# Autodesk Inventor assembly: Łapa
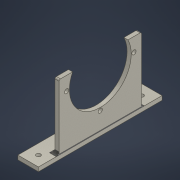
[picture p0: Inventor's stored thumbnail of the model, 180x180]
Saved by Autodesk Inventor 2022 (Build 260153000, 153)
## iProperties
Created: 2023-04-12
Part Number: Łapa
Document SubType Name: Konstrukcja spawana
Designer: jacek
Weld Material: Stal
Author: jacek
## Documents named in this file (3)
- D:\Pulpit\Silownik\Actuator\Łapa.iam
- D:\Pulpit\Silownik\Actuator\łapa2.ipt
- D:\Pulpit\Silownik\Actuator\łapa1.ipt
## Components (2 placed, 2 different names)
1. łapa2:1 — Sztywne:1
2. łapa1:1 — Sztywne:1
## Relationships (1: WeldJoint 1)
- Sztywne:1 [WeldJoint] (1 mm): łapa2:1 ↔ łapa1:1
